# Autodesk Inventor assembly: assy_mission_tunnel
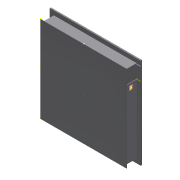
[picture p0: Inventor's stored thumbnail of the model, 180x180]
Saved by Autodesk Inventor 2018 (Build 220112000, 112)
## iProperties
Created: 2017-11-13
Part Number: assy_mission_tunnel
Document SubType Name: Assembly
Designer: Platform
Author: Platform
## Documents named in this file (8)
- C:\Users\Platform\Desktop\autorace_track\track_model\autorace_rbizchallenge2017\assembled\assy_mission_tunnel.iam
- C:\Users\Platform\Desktop\autorace_track\track_model\autorace_rbizchallenge2017\assembled\assy_lower_plates.iam
- C:\Users\Platform\Desktop\autorace_track\track_model\autorace_rbizchallenge2017\parts\ipt\wall_plate_600 v1.ipt
- C:\Users\Platform\Desktop\autorace_track\track_model\autorace_rbizchallenge2017\parts\ipt\wall_plate_910 v1.ipt
- C:\Users\Platform\Desktop\autorace_track\track_model\autorace_rbizchallenge2017\parts\ipt\wall_plate_900 v1.ipt
- C:\Users\Platform\Desktop\autorace_track\track_model\autorace_rbizchallenge2017\parts\ipt\tunnel_line.ipt
- C:\Users\Platform\Desktop\autorace_track\track_model\autorace_rbizchallenge2017\parts\ipt\roof_plate v1.ipt
- C:\Users\Platform\Desktop\autorace_track\track_model\autorace_rbizchallenge2017\parts\ipt\tunnel_sign.ipt
## Components (20 placed, 7 different names)
1. assy_lower_plates:1 [sub-assembly] — Mate:1, Flush:1, Flush:2
2. assy_lower_plates:2 [sub-assembly] — Mate:1, Flush:1, Flush:2, Mate:2, Flush:3, Flush:4
3. assy_lower_plates:3 [sub-assembly] — Mate:2, Flush:3, Flush:4, Mate:3, Mate:4, Flush:5, Mate:5, Mate:6, Flush:6, Mate:7, Mate:9, Mate:13, Flush:10, Flush:11, Mate:14, Mate:16, Mate:18, Mate:20, Flush:14, Mate:22, Flush:15, Mate:24, Flush:16, Mate:26, Flush:17, Mate:29, Mate:30, Mate:38
4. wall_plate_600 v1:1 — Mate:3, Mate:4, Flush:5, Mate:8, Flush:7, Mate:21, Mate:35, Mate:37, Flush:21
5. wall_plate_600 v1:2 — Mate:5, Mate:6, Flush:6, Mate:10, Flush:8, Mate:27, Mate:31
6. wall_plate_910 v1:1 — Mate:7, Mate:8, Flush:7
7. wall_plate_900 v1:1 — Mate:9, Mate:10, Flush:8, Mate:33
8. wall_plate_910 v1:2 — Mate:13, Flush:10, Flush:11, Mate:15, Flush:12, Mate:23
9. wall_plate_910 v1:3 — Mate:14, Mate:15, Flush:12, Mate:17, Flush:22
10. wall_plate_900 v1:3 — Mate:16, Mate:17, Mate:19, Flush:13, Mate:28, Flush:22
11. wall_plate_910 v1:4 — Mate:18, Mate:19, Flush:13, Mate:25
12. tunnel_line:1 — Mate:20, Flush:14, Mate:21
13. tunnel_line:2 — Mate:22, Mate:23, Flush:15
14. tunnel_line:3 — Mate:24, Flush:16, Mate:25
15. tunnel_line:4 — Mate:26, Flush:17, Mate:27
16. roof_plate v1:1 — Mate:28, Mate:29, Mate:30, Flush:18, Mate:32, Flush:20, Mate:36
17. roof_plate v1:2 — Mate:31, Flush:18, Mate:32, Mate:34, Flush:19
18. roof_plate v1:3 — Mate:33, Mate:34, Flush:19
19. roof_plate v1:4 — Mate:35, Flush:20, Mate:36
20. tunnel_sign:1 — Mate:37, Flush:21, Mate:38
## Relationships (57: Mate 36, Flush 21)
- Mate:1: assy_lower_plates:1 ↔ assy_lower_plates:2
- Flush:1: assy_lower_plates:1 ↔ assy_lower_plates:2
- Flush:2: assy_lower_plates:1 ↔ assy_lower_plates:2
- Mate:2: assy_lower_plates:2 ↔ assy_lower_plates:3
- Flush:3: assy_lower_plates:2 ↔ assy_lower_plates:3
- Flush:4: assy_lower_plates:2 ↔ assy_lower_plates:3
- Mate:3: assy_lower_plates:3 ↔ wall_plate_600 v1:1
- Mate:4: assy_lower_plates:3 ↔ wall_plate_600 v1:1
- Flush:5 (90 mm): assy_lower_plates:3 ↔ wall_plate_600 v1:1
- Mate:5: assy_lower_plates:3 ↔ wall_plate_600 v1:2
- Mate:6: assy_lower_plates:3 ↔ wall_plate_600 v1:2
- Flush:6 (90 mm): assy_lower_plates:3 ↔ wall_plate_600 v1:2
- Mate:7: assy_lower_plates:3 ↔ wall_plate_910 v1:1
- Mate:8: wall_plate_600 v1:1 ↔ wall_plate_910 v1:1
- Flush:7: wall_plate_600 v1:1 ↔ wall_plate_910 v1:1
- Mate:9: assy_lower_plates:3 ↔ wall_plate_900 v1:1
- Mate:10: wall_plate_600 v1:2 ↔ wall_plate_900 v1:1
- Flush:8: wall_plate_600 v1:2 ↔ wall_plate_900 v1:1
- Mate:13: assy_lower_plates:3 ↔ wall_plate_910 v1:2
- Flush:10 (90 mm): assy_lower_plates:3 ↔ wall_plate_910 v1:2
- Flush:11 (90 mm): assy_lower_plates:3 ↔ wall_plate_910 v1:2
- Mate:14: assy_lower_plates:3 ↔ wall_plate_910 v1:3
- Mate:15: wall_plate_910 v1:2 ↔ wall_plate_910 v1:3
- Flush:12: wall_plate_910 v1:2 ↔ wall_plate_910 v1:3
- Mate:16: assy_lower_plates:3 ↔ wall_plate_900 v1:3
- Mate:17: wall_plate_910 v1:3 ↔ wall_plate_900 v1:3
- Mate:18: assy_lower_plates:3 ↔ wall_plate_910 v1:4
- Mate:19: wall_plate_900 v1:3 ↔ wall_plate_910 v1:4
- Flush:13: wall_plate_900 v1:3 ↔ wall_plate_910 v1:4
- Mate:20: assy_lower_plates:3 ↔ tunnel_line:1
- Flush:14: assy_lower_plates:3 ↔ tunnel_line:1
- Mate:21: wall_plate_600 v1:1 ↔ tunnel_line:1
- Mate:22: assy_lower_plates:3 ↔ tunnel_line:2
- Mate:23: wall_plate_910 v1:2 ↔ tunnel_line:2
- Flush:15: assy_lower_plates:3 ↔ tunnel_line:2
- Mate:24: assy_lower_plates:3 ↔ tunnel_line:3
- Flush:16: assy_lower_plates:3 ↔ tunnel_line:3
- Mate:25: wall_plate_910 v1:4 ↔ tunnel_line:3
- Mate:26: assy_lower_plates:3 ↔ tunnel_line:4
- Flush:17: assy_lower_plates:3 ↔ tunnel_line:4
- Mate:27: wall_plate_600 v1:2 ↔ tunnel_line:4
- Mate:28: wall_plate_900 v1:3 ↔ roof_plate v1:1
- Mate:29: assy_lower_plates:3 ↔ roof_plate v1:1
- Mate:30: assy_lower_plates:3 ↔ roof_plate v1:1
- Mate:31: wall_plate_600 v1:2 ↔ roof_plate v1:2
- Flush:18: roof_plate v1:1 ↔ roof_plate v1:2
- Mate:32: roof_plate v1:1 ↔ roof_plate v1:2
- Mate:33: wall_plate_900 v1:1 ↔ roof_plate v1:3
- Mate:34: roof_plate v1:2 ↔ roof_plate v1:3
- Flush:19: roof_plate v1:2 ↔ roof_plate v1:3
- Mate:35: wall_plate_600 v1:1 ↔ roof_plate v1:4
- Flush:20: roof_plate v1:1 ↔ roof_plate v1:4
- Mate:36: roof_plate v1:1 ↔ roof_plate v1:4
- Mate:37: wall_plate_600 v1:1 ↔ tunnel_sign:1
- Flush:21 (50 mm): wall_plate_600 v1:1 ↔ tunnel_sign:1
- Mate:38 (80 mm): assy_lower_plates:3 ↔ tunnel_sign:1
- Flush:22: wall_plate_910 v1:3 ↔ wall_plate_900 v1:3
